# Autodesk Inventor assembly: Toughbox-mini
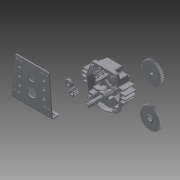
[picture p0: Inventor's stored thumbnail of the model, 180x180]
Saved by Autodesk Inventor 2014 SP1 (Build 180222100, 222)
## iProperties
Created: 2014-01-17
Part Number: Toughbox-mini
Document SubType Name: Assembly
Designer: Paul
Author: Paul
Author: Unknown
Title: S:/Products/Gearboxes Spur Single Stage/Toughbox/Toughbox Mini/Toughbox-Mini.stp
Organization: Unknown
Description: Unknown
Sending System: Unknown
Preprocessor: XStep 1.0
## Documents named in this file (15)
- C:\FRC_CAD\4859cad\Robot\Drivetrain\Drivetrain Assembly\Imported Components\Toughbox-mini\Toughbox-mini.iam
- C:\FRC_CAD\4859cad\Robot\Drivetrain\Drivetrain Assembly\Imported Components\Toughbox-mini\r6zz.ipt
- C:\FRC_CAD\4859cad\Robot\Drivetrain\Drivetrain Assembly\Imported Components\Toughbox-mini\Toughbox_d07.ipt
- C:\FRC_CAD\4859cad\Robot\Drivetrain\Drivetrain Assembly\Imported Components\Toughbox-mini\Toughbox_d05.ipt
- C:\FRC_CAD\4859cad\Robot\Drivetrain\Drivetrain Assembly\Imported Components\Toughbox-mini\Toughbox_d08.ipt
- C:\FRC_CAD\4859cad\Robot\Drivetrain\Drivetrain Assembly\Imported Components\Toughbox-mini\Toughbox_d06.ipt
- C:\FRC_CAD\4859cad\Robot\Drivetrain\Drivetrain Assembly\Imported Components\Toughbox-mini\fr-6-zz.ipt
- C:\FRC_CAD\4859cad\Robot\Drivetrain\Drivetrain Assembly\Imported Components\Toughbox-mini\fr-8-zz.ipt
- C:\FRC_CAD\4859cad\Robot\Drivetrain\Drivetrain Assembly\Imported Components\Toughbox-mini\10-32_nylock_nut.ipt
- C:\FRC_CAD\4859cad\Robot\Drivetrain\Drivetrain Assembly\Imported Components\Toughbox-mini\5-16_washer.ipt
- C:\FRC_CAD\4859cad\Robot\Drivetrain\Drivetrain Assembly\Imported Components\Toughbox-mini\Toughbox_d09.ipt
- C:\FRC_CAD\4859cad\Robot\Drivetrain\Drivetrain Assembly\Imported Components\Toughbox-mini\8mm_spring_clip.ipt
- C:\FRC_CAD\4859cad\Robot\Drivetrain\Drivetrain Assembly\Imported Components\Toughbox-mini\Toughbox-mini_d01-5-12.ipt
- C:\FRC_CAD\4859cad\Robot\Drivetrain\Drivetrain Assembly\Imported Components\Toughbox-mini\Toughbox-mini_d02.ipt
- C:\FRC_CAD\4859cad\Robot\Drivetrain\Drivetrain Assembly\Imported Components\Toughbox-mini\10-32x0625_shcs.ipt
## Components (30 placed, 14 different names)
1. r6zz — Mate:1, Mate:2, Mate:3, Mate:4, Mate:5
2. r6zz:1
3. Toughbox_d07 — Mate:3, Mate:4, Mate:6, Mate:7, Mate:9, Mate:10, Mate:11
4. Toughbox_d05 — Mate:5, Mate:6, Mate:7, Mate:8
5. Toughbox_d08 — Mate:8, Mate:9, Mate:10, Mate:12
6. Toughbox_d06
7. fr-6-zz — Mate:11, Mate:12
8. fr-8-zz
9. 10-32_nylock_nut
10. 10-32_nylock_nut:1
11. 10-32_nylock_nut:2
12. 10-32_nylock_nut:3
13. 5-16_washer
14. 5-16_washer:1
15. 5-16_washer:2
16. 5-16_washer:3
17. Toughbox_d09
18. Toughbox_d09:1
19. 8mm_spring_clip
20. 8mm_spring_clip:1
21. Toughbox-mini_d01-5-12 — Mate:1, Mate:2
22. Toughbox-mini_d02
23. 10-32x0625_shcs
24. 10-32x0625_shcs:1
25. 10-32x0625_shcs:2
26. 10-32x0625_shcs:3
27. 10-32x0625_shcs:4
28. 10-32x0625_shcs:5
29. 10-32x0625_shcs:6
30. 10-32x0625_shcs:7
## Relationships (12: Mate 12)
- Mate:1: r6zz ↔ Toughbox-mini_d01-5-12
- Mate:2: r6zz ↔ Toughbox-mini_d01-5-12
- Mate:3: r6zz ↔ Toughbox_d07
- Mate:4: r6zz ↔ Toughbox_d07
- Mate:5: r6zz ↔ Toughbox_d05
- Mate:6: Toughbox_d07 ↔ Toughbox_d05
- Mate:7: Toughbox_d07 ↔ Toughbox_d05
- Mate:8: Toughbox_d05 ↔ Toughbox_d08
- Mate:9: Toughbox_d07 ↔ Toughbox_d08
- Mate:10: Toughbox_d07 ↔ Toughbox_d08
- Mate:11: Toughbox_d07 ↔ fr-6-zz
- Mate:12: Toughbox_d08 ↔ fr-6-zz
